# Autodesk Inventor assembly: SchlittenUnten
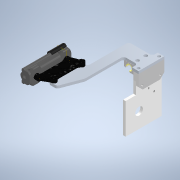
[picture p0: Inventor's stored thumbnail of the model, 180x180]
Saved by Autodesk Inventor 2022 (Build 260153000, 153)
## iProperties
Created: 2022-03-23
Part Number: SchlittenUnten
Document SubType Name: Assembly
Designer: kaebi
Author: kaebi
## Documents named in this file (6)
- C:\Users\kaebi\OneDrive - mci4me.at\03_MCI Master\4.Semester_SS2022\Masterarbeit\Software\CAD\106_Vereinzelungseinheit\SchlittenUnten.iam
- C:\Users\kaebi\OneDrive - mci4me.at\03_MCI Master\4.Semester_SS2022\Masterarbeit\Software\CAD\106_Vereinzelungseinheit\106.016.01_Schienenfuehrung.ipt
- C:\Users\kaebi\OneDrive - mci4me.at\03_MCI Master\4.Semester_SS2022\Masterarbeit\Software\CAD\106_Vereinzelungseinheit\106.034.01_Schieberelement_unten.ipt
- C:\Users\kaebi\OneDrive - mci4me.at\03_MCI Master\4.Semester_SS2022\Masterarbeit\Software\CAD\106_Vereinzelungseinheit\106.020.01_Winkelaufnahme_Schwert_unten.ipt
- C:\Users\kaebi\OneDrive - mci4me.at\03_MCI Master\4.Semester_SS2022\Masterarbeit\Software\CAD\106_Vereinzelungseinheit\106.033.01_Schwert_unten.ipt
- C:\Users\kaebi\OneDrive - mci4me.at\03_MCI Master\4.Semester_SS2022\Masterarbeit\Software\CAD\106_Vereinzelungseinheit\206.003.02_Kraftlimitierung.iam
## Components (6 placed, 5 different names)
1. 106.016.01_Schienenfuehrung:1 — Passend:15
2. 106.016.01_Schienenfuehrung:3 — Passend:13, Passend:14
3. 106.034.01_Schieberelement_unten:1 — Passend:13, Passend:14, Passend:15
4. 106.020.01_Winkelaufnahme_Schwert_unten:1
5. 106.033.01_Schwert_unten:1
6. 206.003.02_Kraftlimitierung:1 [sub-assembly]
## Relationships (15: Mate 15)
- [Mate]: 106.016.01_Schienenfuehrung:3 ↔ 106.034.01_Schieberelement_unten:1
- [Mate]: 106.016.01_Schienenfuehrung:1 ↔ 106.034.01_Schieberelement_unten:1
- [Mate]: 106.034.01_Schieberelement_unten:1 ↔ 106.020.01_Winkelaufnahme_Schwert_unten:1
- [Mate]: 106.034.01_Schieberelement_unten:1 ↔ 106.020.01_Winkelaufnahme_Schwert_unten:1
- [Mate]: 106.034.01_Schieberelement_unten:1 ↔ 106.020.01_Winkelaufnahme_Schwert_unten:1
- [Mate]: 106.020.01_Winkelaufnahme_Schwert_unten:1 ↔ 106.033.01_Schwert_unten:1
- [Mate]: 106.020.01_Winkelaufnahme_Schwert_unten:1 ↔ 106.033.01_Schwert_unten:1
- [Mate]: 106.020.01_Winkelaufnahme_Schwert_unten:1 ↔ 106.033.01_Schwert_unten:1
- [Mate]: 106.034.01_Schieberelement_unten:1 ↔ 206.003.02_Kraftlimitierung:1
- [Mate]: 106.016.01_Schienenfuehrung:1 ↔ 106.034.01_Schieberelement_unten:1
- [Mate]: 106.034.01_Schieberelement_unten:1 ↔ 206.003.02_Kraftlimitierung:1
- [Mate]: 106.034.01_Schieberelement_unten:1 ↔ 206.003.02_Kraftlimitierung:1
- Passend:13 [Mate]: 106.016.01_Schienenfuehrung:3 ↔ 106.034.01_Schieberelement_unten:1
- Passend:14 [Mate]: 106.016.01_Schienenfuehrung:3 ↔ 106.034.01_Schieberelement_unten:1
- Passend:15 [Mate]: 106.016.01_Schienenfuehrung:1 ↔ 106.034.01_Schieberelement_unten:1
